# Autodesk Inventor assembly: Robot
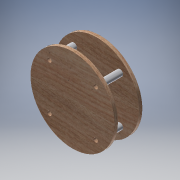
[picture p0: Inventor's stored thumbnail of the model, 180x180]
Saved by Autodesk Inventor 2017.3 (Build 213256000, 256)
## iProperties
Part Number: Robot
Material: Générique
Document SubType Name: Assembly
Designer: Piou piou
Author: Piou piou
## Documents named in this file (5)
- D:\Documents\cours polytech\projet slam\robot\Robot.iam
- D:\Documents\cours polytech\projet slam\robot\dessus.ipt
- D:\Documents\cours polytech\projet slam\robot\Servomoteur HS-311.ipt
- D:\Documents\cours polytech\projet slam\robot\base.ipt
- D:\Documents\cours polytech\projet slam\robot\tube.ipt
## Components (7 placed, 4 different names)
1. dessus:1 — Placage:1, Placage:2, Placage:3, Placage:4, Placage:13, Placage:14, Placage:15
2. Servomoteur HS-311:1 — Placage:1, Placage:2, Placage:3, Placage:4
3. base:1 — Placage:5, Placage:6, Placage:7, Placage:8, Placage:9, Placage:10, Placage:11, Placage:12
4. tube:1 — Placage:5, Placage:11
5. tube:2 — Placage:6, Placage:12, Placage:15
6. tube:4 — Placage:8, Placage:9, Placage:13
7. tube:5 — Placage:7, Placage:10, Placage:14
## Relationships (15: Mate 15)
- Placage:1 [Mate]: dessus:1 ↔ Servomoteur HS-311:1
- Placage:2 [Mate]: dessus:1 ↔ Servomoteur HS-311:1
- Placage:3 [Mate]: dessus:1 ↔ Servomoteur HS-311:1
- Placage:4 [Mate]: dessus:1 ↔ Servomoteur HS-311:1
- Placage:5 [Mate]: base:1 ↔ tube:1
- Placage:6 [Mate]: base:1 ↔ tube:2
- Placage:7 [Mate]: base:1 ↔ tube:5
- Placage:8 [Mate]: base:1 ↔ tube:4
- Placage:9 [Mate]: base:1 ↔ tube:4
- Placage:10 [Mate]: base:1 ↔ tube:5
- Placage:11 [Mate]: base:1 ↔ tube:1
- Placage:12 [Mate]: base:1 ↔ tube:2
- Placage:13 [Mate]: dessus:1 ↔ tube:4
- Placage:14 [Mate]: dessus:1 ↔ tube:5
- Placage:15 [Mate]: dessus:1 ↔ tube:2
